# Autodesk Inventor assembly: Complet
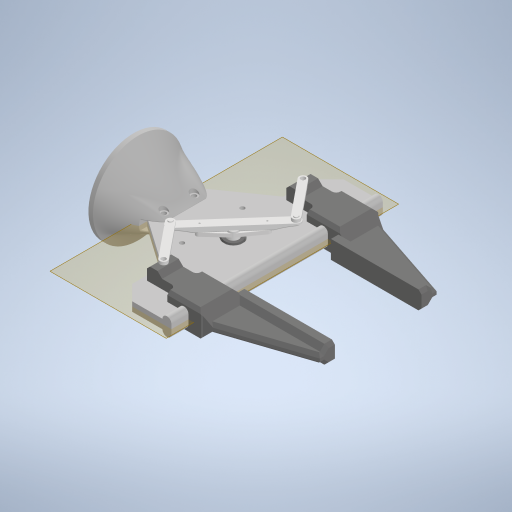
[picture p0: Inventor's stored thumbnail of the model, 512x512]
Saved by Autodesk Inventor 2023 (Build 270158000, 158)
## iProperties
Created: 2024-07-03
Part Number: Complet
Document SubType Name: Assembly
Designer: Swoby
Author: Swoby
## Documents named in this file (8)
- C:\Users\Swoby\OneDrive\Plocha\DUM-E\V0.3\Complet.iam
- C:\Users\Swoby\OneDrive\Plocha\DUM-E\V0.3\gripper_head 1.ipt
- C:\Users\Swoby\OneDrive\Plocha\DUM-E\V0.3\gripper_head 2.ipt
- C:\Users\Swoby\OneDrive\Plocha\DUM-E\V0.3\gripper_gripper.ipt
- C:\Users\Swoby\OneDrive\Plocha\DUM-E\V0.3\gripper_mechanism.ipt
- C:\Users\Swoby\OneDrive\Plocha\DUM-E\V0.3\gripper_mechanism2.ipt
- C:\Users\Swoby\OneDrive\Plocha\DUM-E\V0.3\Servo_small_top.ipt
- C:\Users\Swoby\OneDrive\Plocha\DUM-E\V0.3\Servo_small_maketa.ipt
## Components (9 placed, 7 different names)
1. gripper_head 1:1 — Mate:1, Mate:2, Mate:3, Mate:4, Mate:5, Mate:6, Mate:7, Mate:8, Mate:9, Mate:10
2. gripper_head 2:1 — Mate:1, Mate:2, Mate:3
3. gripper_gripper:1 — Mate:4, Mate:7, Mate:18
4. gripper_gripper:2 — Mate:5, Mate:6, Mate:20
5. gripper_mechanism:1 — Mate:13, Mate:14, Mate:15, Mate:16, Mate:17, Mate:19, Mate:21, Mate:22, Mate:23
6. gripper_mechanism2:1 — Mate:16, Mate:17, Mate:18, Mate:22
7. gripper_mechanism2:2 — Mate:19, Mate:20, Mate:21, Mate:23
8. Servo_small_top:1 — Mate:11, Mate:12, Mate:13, Mate:14, Mate:15
9. Servo_small_maketa:1 — Mate:8, Mate:9, Mate:10, Mate:11, Mate:12
## Relationships (23: Mate 23)
- Mate:1: gripper_head 1:1 ↔ gripper_head 2:1
- Mate:2: gripper_head 1:1 ↔ gripper_head 2:1
- Mate:3: gripper_head 1:1 ↔ gripper_head 2:1
- Mate:4: gripper_head 1:1 ↔ gripper_gripper:1
- Mate:5: gripper_head 1:1 ↔ gripper_gripper:2
- Mate:6: gripper_head 1:1 ↔ gripper_gripper:2
- Mate:7: gripper_head 1:1 ↔ gripper_gripper:1
- Mate:8: gripper_head 1:1 ↔ Servo_small_maketa:1
- Mate:9: gripper_head 1:1 ↔ Servo_small_maketa:1
- Mate:10: gripper_head 1:1 ↔ Servo_small_maketa:1
- Mate:11: Servo_small_top:1 ↔ Servo_small_maketa:1
- Mate:12: Servo_small_top:1 ↔ Servo_small_maketa:1
- Mate:13: gripper_mechanism:1 ↔ Servo_small_top:1
- Mate:14: gripper_mechanism:1 ↔ Servo_small_top:1
- Mate:15: gripper_mechanism:1 ↔ Servo_small_top:1
- Mate:16: gripper_mechanism:1 ↔ gripper_mechanism2:1
- Mate:17: gripper_mechanism:1 ↔ gripper_mechanism2:1
- Mate:18: gripper_gripper:1 ↔ gripper_mechanism2:1
- Mate:19: gripper_mechanism:1 ↔ gripper_mechanism2:2
- Mate:20: gripper_gripper:2 ↔ gripper_mechanism2:2
- Mate:21: gripper_mechanism:1 ↔ gripper_mechanism2:2
- Mate:22: gripper_mechanism:1 ↔ gripper_mechanism2:1
- Mate:23: gripper_mechanism:1 ↔ gripper_mechanism2:2
